# Autodesk Inventor assembly: Delivery bin inside arm
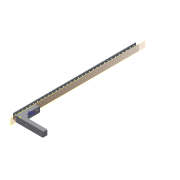
[picture p0: Inventor's stored thumbnail of the model, 180x180]
Saved by Autodesk Inventor 2018 (Build 220112000, 112)
## iProperties
Created: 2019-01-05
Part Number: Delivery bin inside arm
Document SubType Name: Assembly
Designer: ball
Author: ball
## Documents named in this file (3)
- C:\FTC\FTC8863CAD\2018Robot\Delivery bin inside arm.iam
- C:\FTC\FTC8863CAD\Actobotics\585 parts\585399.ipt
- C:\FTC\FTC8863CAD\2018Robot\Delivery bin right angle connector.ipt
## Components (2 placed, 2 different names)
1. 585399:1 — Flush:1
2. Delivery bin right angle connector:1 — Flush:1
## Relationships (1: Flush 1)
- Flush:1: 585399:1 ↔ Delivery bin right angle connector:1
